# Autodesk Inventor assembly: Подшипниковый блок поворотного узла манипулятора
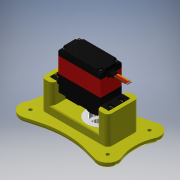
[picture p0: Inventor's stored thumbnail of the model, 180x180]
Saved by Autodesk Inventor 2019.1 (Build 231200000, 200)
## iProperties
Created: 2018-10-15
Part Number: Подшипниковый блок поворотного узла манипулятора
Material: Типовые
Document SubType Name: Assembly
Designer: Олег
Author: Олег
## Documents named in this file (4)
- C:\Users\Олег\OneDrive\Общая\NoSpace 2.0\Манипулятор\Поворотный узел манипулятора\Поворотный узел манипулятора.iam
- C:\Users\Олег\OneDrive\Общая\NoSpace 2.0\Манипулятор\PDI 6621MG.ipt
- C:\Users\Олег\OneDrive\Общая\NoSpace 2.0\Манипулятор\Поворотный узел манипулятора\Блок подшипника поворотного узла манипулятора.ipt
- C:\Users\Олег\OneDrive\Общая\NoSpace 2.0\Манипулятор\Поворотный узел манипулятора\Подшипник 17х26х5.ipt
## Components (4 placed, 3 different names)
1. PDI 6621MG:1 — Совмещение:4, Совмещение:5, Совмещение:6
2. Блок подшипника поворотного узла манипулятора:1 — Совмещение:1, Заподлицо:1, Совмещение:3, Совмещение:4, Совмещение:5, Совмещение:6
3. Подшипник 17х26х5:1 — Совмещение:1, Заподлицо:1, Совмещение:2
4. Подшипник 17х26х5:2 — Совмещение:2, Совмещение:3
## Relationships (7: Mate 6, Flush 1)
- Совмещение:1 [Mate]: Блок подшипника поворотного узла манипулятора:1 ↔ Подшипник 17х26х5:1
- Заподлицо:1 [Flush]: Блок подшипника поворотного узла манипулятора:1 ↔ Подшипник 17х26х5:1
- Совмещение:2 [Mate]: Подшипник 17х26х5:1 ↔ Подшипник 17х26х5:2
- Совмещение:3 [Mate]: Блок подшипника поворотного узла манипулятора:1 ↔ Подшипник 17х26х5:2
- Совмещение:4 [Mate]: PDI 6621MG:1 ↔ Блок подшипника поворотного узла манипулятора:1
- Совмещение:5 [Mate]: PDI 6621MG:1 ↔ Блок подшипника поворотного узла манипулятора:1
- Совмещение:6 [Mate]: PDI 6621MG:1 ↔ Блок подшипника поворотного узла манипулятора:1
